# Autodesk Inventor assembly: Acrylic Housing
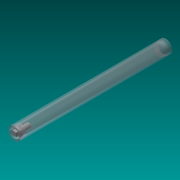
[picture p0: Inventor's stored thumbnail of the model, 180x180]
Saved by Autodesk Inventor 2015 (Build 190159000, 159)
## iProperties
Created: 2015-01-31
Part Number: Acrylic Housing
Document SubType Name: Assembly
Designer: Sawaiz Syed
Author: Sawaiz Syed
## Documents named in this file (5)
- C:\Users\Admin\SkyDrive\Classes\Reaserch\RadiationSensor\Hardware\Transmitter 3D\Inventor\Radiation Dector\Acrylic Housing.iam
- C:\Users\Admin\SkyDrive\Classes\Reaserch\RadiationSensor\Hardware\Transmitter 3D\Inventor\Radiation Dector\Acrylic Tube Housing.ipt
- C:\Users\Admin\SkyDrive\Classes\Reaserch\RadiationSensor\Hardware\Transmitter 3D\Inventor\Radiation Dector\Back Cap.ipt
- C:\Users\Admin\SkyDrive\Classes\Reaserch\RadiationSensor\Hardware\Transmitter 3D\Inventor\Radiation Dector\Switch Cap.ipt
- C:\Users\Admin\SkyDrive\Classes\Reaserch\RadiationSensor\Hardware\Transmitter 3D\Inventor\Radiation Dector\Power Switch.ipt
## Components (4 placed, 4 different names)
1. Acrylic Tube Housing:1 — Rigid:1, Rigid:2
2. Back Cap:1 — Rigid:1
3. Switch Cap:1 — Rigid:2, Mate:1, Mate:2
4. Power Switch:1 — Mate:1, Mate:2
## Relationships (4: WeldJoint 2, Mate 2)
- Rigid:1 [WeldJoint]: Acrylic Tube Housing:1 ↔ Back Cap:1
- Rigid:2 [WeldJoint]: Acrylic Tube Housing:1 ↔ Switch Cap:1
- Mate:1: Switch Cap:1 ↔ Power Switch:1
- Mate:2: Switch Cap:1 ↔ Power Switch:1
